# Autodesk Inventor assembly: singleModule
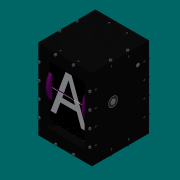
[picture p0: Inventor's stored thumbnail of the model, 180x180]
Saved by Autodesk Inventor 2016 (Build 200138000, 138)
## iProperties
Created: 2015-10-05
Part Number: singleModule
Document SubType Name: Assembly
Designer: Sawaiz
Author: Sawaiz
## Documents named in this file (10)
- C:\Users\sawai\OneDrive\projects\splitFlapDisplay\singleModule.iam
- C:\Users\sawai\OneDrive\projects\splitFlapDisplay\frame\frame.iam
- C:\Users\sawai\OneDrive\projects\splitFlapDisplay\spool\cardSpool.iam
- C:\Users\sawai\OneDrive\projects\splitFlapDisplay\drive\drive.iam
- C:\Users\sawai\OneDrive\projects\splitFlapDisplay\drive\gt236Tooth.ipt
- C:\Users\sawai\OneDrive\projects\splitFlapDisplay\drive\axleSpacer.ipt
- C:\Users\sawai\OneDrive\projects\splitFlapDisplay\drive\centeralShaft.ipt
- C:\Users\sawai\OneDrive\projects\splitFlapDisplay\drive\belt.ipt
- C:\Users\sawai\OneDrive\projects\splitFlapDisplay\frame\608RS.ipt
- C:\Users\sawai\OneDrive\projects\splitFlapDisplay\parameters.xlsx
## Components (9 placed, 8 different names)
1. cardSpool:1 [sub-assembly] — Mate:10, Angle:1, Mate:11, Mate:12, Mate:13
2. drive:1 [sub-assembly] — Flush:1, Mate:7, Mate:8, Mate:9, Mate:19
3. gt236Tooth:1 — Flush:1, Mate:18, Mate:20
4. frame:1 [sub-assembly] — Mate:7, Mate:8, Mate:9, Mate:10, Angle:1, Mate:11, Mate:14, Flush:2, Mate:18, Angle:2, Flush:3
5. axleSpacer:1 — Mate:12, Mate:13
6. centeralShaft:1 — Mate:14, Flush:2
7. 608RS:1 — Mate:21, Mate:22
8. belt:1 — Mate:19, Angle:2, Mate:20, Mate:21
9. centeralShaft:2 — Mate:22, Flush:3
## Relationships (18: Mate 13, Flush 3, Angle 2)
- Flush:1: drive:1 ↔ gt236Tooth:1
- Mate:7: drive:1 ↔ frame:1
- Mate:8: drive:1 ↔ frame:1
- Mate:9: drive:1 ↔ frame:1
- Mate:10: cardSpool:1 ↔ frame:1
- Angle:1 (0 deg): cardSpool:1 ↔ frame:1
- Mate:11 (0.5 mm): cardSpool:1 ↔ frame:1
- Mate:12: cardSpool:1 ↔ axleSpacer:1
- Mate:13: cardSpool:1 ↔ axleSpacer:1
- Mate:14: frame:1 ↔ centeralShaft:1
- Flush:2: frame:1 ↔ centeralShaft:1
- Mate:18: gt236Tooth:1 ↔ frame:1
- Mate:19: drive:1 ↔ belt:1
- Angle:2 (0 deg): frame:1 ↔ belt:1
- Mate:20 (0.5 mm): gt236Tooth:1 ↔ belt:1
- Mate:21: 608RS:1 ↔ belt:1
- Mate:22: 608RS:1 ↔ centeralShaft:2
- Flush:3: frame:1 ↔ centeralShaft:2
## Named parameters: height = 180 mm, width = 120 mm, depth = 115 mm, materialThickness = 6.35 mm, laserKerf = 0.1 mm, spoolDiameter = 95 mm, cardPinDiameter = 3 mm, cardNumber = 40, centeralShaftDiameter = 8 mm, cardWidth = 85.6 mm, cardHeight = 53.98 mm, cardThickness = 0.76 mm, cardFillet = 2.88 mm, cardCutoutHeight = 20 mm, cardClearence = 0.5 mm, spoolHubDiameter = 20 mm, bearingOd = 22 mm, bearingWidth = 8 mm, axleHeight = 95 mm, nutTrapDepth = 2.5 mm, nutTrapwidth = 5.5 mm, nutTrapClearence = 2 mm, beltLength = 350 mm
